# Autodesk Inventor assembly: Reload_Assembly
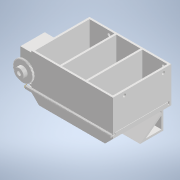
[picture p0: Inventor's stored thumbnail of the model, 180x180]
Saved by Autodesk Inventor 2020 (Build 240168000, 168)
## iProperties
Created: 2022-03-20
Part Number: Reload_Assembly
Document SubType Name: Assembly
Designer: danie
Author: danie
## Documents named in this file (5)
- C:\Users\danie\Documents\Capstone\Solidworks\Reload_Assembly.iam
- C:\Users\danie\Documents\Capstone\Solidworks\BeadCompartments_5.ipt
- C:\Users\danie\Documents\Capstone\Solidworks\Reload_Motor.ipt
- C:\Users\danie\Documents\Capstone\Solidworks\False_Bottom_Geared_2.iam
- C:\Users\danie\Documents\Capstone\Solidworks\ShootingMech_ReloadGear.ipt
## Components (4 placed, 4 different names)
1. BeadCompartments_5:1 — Rigid:1
2. Reload_Motor:1 — Rotational:1
3. False_Bottom_Geared_2:1 [sub-assembly] — Rigid:1
4. ShootingMech_ReloadGear:1 — Rotational:1
## Relationships (2: WeldJoint 1, RevoluteJoint 1)
- Rigid:1 [WeldJoint] (3.81 mm): BeadCompartments_5:1 ↔ False_Bottom_Geared_2:1
- Rotational:1 [RevoluteJoint]: Reload_Motor:1 ↔ ShootingMech_ReloadGear:1
